# Autodesk Inventor assembly: Swerve-Drivetrain-2
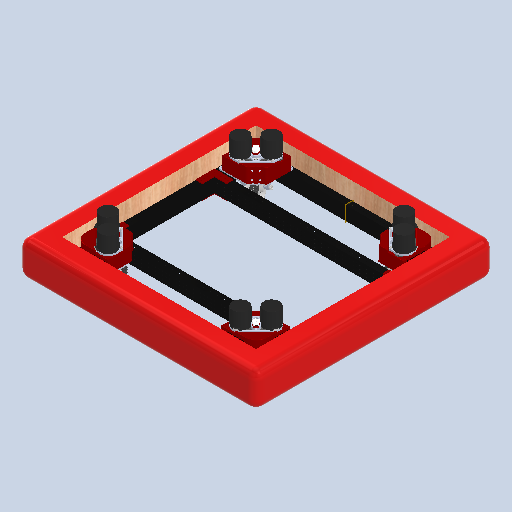
[picture p0: Inventor's stored thumbnail of the model, 512x512]
Saved by Autodesk Inventor 2024 (Build 280153000, 153)
## iProperties
Created: 2024-01-06
Part Number: Swerve-Drivetrain-2
Document SubType Name: Assembly
Designer: rohan
Author: rohan
## Documents named in this file (7)
- C:\Users\5652160\OneDrive - Hillsborough County Public Schools\Robotics\FIRST-Robotics-Competition\Crescendo\Minotaur-Crescendo-Robot\Swerve-Drivetrain.iam
- C:\Users\5652160\OneDrive - Hillsborough County Public Schools\Robotics\FIRST-Robotics-Competition\Crescendo\Minotaur-Crescendo-Robot\Motion\Swerve-Modules\MK3-Swerve-Module-Neos.iam
- C:\Users\5652160\OneDrive - Hillsborough County Public Schools\Robotics\FIRST-Robotics-Competition\Crescendo\Minotaur-Crescendo-Robot\Structure\MAXTube\2024-100-002-Front-Back-Extrusions.ipt
- C:\Users\5652160\OneDrive - Hillsborough County Public Schools\Robotics\FIRST-Robotics-Competition\Crescendo\Minotaur-Crescendo-Robot\Structure\MAXTube\2024-100-001-Left-Right-Extrusions.ipt
- C:\Users\5652160\OneDrive - Hillsborough County Public Schools\Robotics\FIRST-Robotics-Competition\Crescendo\Minotaur-Crescendo-Robot\Structure\MAXTube\2024-100-003-Middle-Extrusions.ipt
- C:\Users\5652160\OneDrive - Hillsborough County Public Schools\Robotics\FIRST-Robotics-Competition\Crescendo\Minotaur-Crescendo-Robot\Structure\Gussets\THRIFYBOT-L-Gusset.ipt
- C:\Users\5652160\OneDrive - Hillsborough County Public Schools\Robotics\FIRST-Robotics-Competition\Crescendo\Minotaur-Crescendo-Robot\Structure\Bumpers.ipt
## Components (23 placed, 6 different names)
1. MK3-Swerve-Module-Neos:1 [sub-assembly] — Mate:75, Mate:80, Mate:81
2. MK3-Swerve-Module-Neos:2 [sub-assembly] — Mate:74, Mate:82, Mate:83
3. MK3-Swerve-Module-Neos:3 [sub-assembly] — Mate:73, Mate:76, Mate:77
4. MK3-Swerve-Module-Neos:4 [sub-assembly] — Mate:72, Mate:78, Mate:79
5. 2024-100-001-Left-Right-Extrusions:1 — Mate:69, Flush:1, Flush:2, Mate:70, Flush:3, Flush:4, Mate:73, Mate:76, Mate:82, Flush:12, Flush:14
6. 2024-100-001-Left-Right-Extrusions:2 — Mate:71, Flush:5, Flush:6, Mate:79, Mate:81, Flush:10, Flush:16, Mate:99
7. 2024-100-002-Front-Back-Extrusions:1 — Mate:70, Flush:3, Flush:4, Mate:72, Mate:77, Mate:78, Mate:84, Mate:85, Mate:88, Mate:89, Flush:13, Flush:15, Flush:30, Mate:96, Flush:32, Mate:97, Flush:33
8. 2024-100-002-Front-Back-Extrusions:2 — Mate:69, Flush:1, Flush:2, Mate:71, Flush:5, Flush:6, Mate:74, Mate:75, Mate:80, Mate:83, Flush:7, Flush:8, Mate:86, Mate:87, Flush:9, Flush:11, Flush:25, Mate:94, Flush:27, Mate:95, Insert:1, Insert:2, Mate:98
9. 2024-100-003-Middle-Extrusions:1 — Mate:85, Flush:7, Flush:26, Flush:29
10. 2024-100-003-Middle-Extrusions:2 — Mate:84, Flush:8, Flush:28, Flush:31
11. THRIFYBOT-L-Gusset:1 — Mate:89, Flush:13, Flush:14
12. THRIFYBOT-L-Gusset:2 — Mate:88, Flush:15, Flush:16
13. THRIFYBOT-L-Gusset:3 — Mate:87, Flush:11, Flush:12
14. THRIFYBOT-L-Gusset:4 — Mate:86, Flush:9, Flush:10
15. THRIFYBOT-L-Gusset:6 — Flush:17, Flush:18, Mate:90, Flush:25, Mate:94, Flush:26, Insert:1
16. THRIFYBOT-L-Gusset:7 — Flush:17, Flush:18, Mate:90
17. THRIFYBOT-L-Gusset:8 — Flush:27, Flush:28, Insert:2
18. THRIFYBOT-L-Gusset:9 — Mate:95
19. THRIFYBOT-L-Gusset:10 — Flush:29, Flush:30
20. THRIFYBOT-L-Gusset:11 — Mate:96
21. THRIFYBOT-L-Gusset:12 — Flush:32, Mate:97
22. THRIFYBOT-L-Gusset:13 — Flush:31
23. Bumpers:1 — Mate:98, Mate:99, Flush:33
## Relationships (66: Flush 33, Mate 31, Insert 2)
- Mate:69: 2024-100-001-Left-Right-Extrusions:1 ↔ 2024-100-002-Front-Back-Extrusions:2
- Flush:1: 2024-100-001-Left-Right-Extrusions:1 ↔ 2024-100-002-Front-Back-Extrusions:2
- Flush:2: 2024-100-001-Left-Right-Extrusions:1 ↔ 2024-100-002-Front-Back-Extrusions:2
- Mate:70: 2024-100-001-Left-Right-Extrusions:1 ↔ 2024-100-002-Front-Back-Extrusions:1
- Flush:3: 2024-100-001-Left-Right-Extrusions:1 ↔ 2024-100-002-Front-Back-Extrusions:1
- Flush:4: 2024-100-001-Left-Right-Extrusions:1 ↔ 2024-100-002-Front-Back-Extrusions:1
- Mate:71: 2024-100-001-Left-Right-Extrusions:2 ↔ 2024-100-002-Front-Back-Extrusions:2
- Flush:5: 2024-100-001-Left-Right-Extrusions:2 ↔ 2024-100-002-Front-Back-Extrusions:2
- Flush:6: 2024-100-001-Left-Right-Extrusions:2 ↔ 2024-100-002-Front-Back-Extrusions:2
- Mate:72: MK3-Swerve-Module-Neos:4 ↔ 2024-100-002-Front-Back-Extrusions:1
- Mate:73: MK3-Swerve-Module-Neos:3 ↔ 2024-100-001-Left-Right-Extrusions:1
- Mate:74: MK3-Swerve-Module-Neos:2 ↔ 2024-100-002-Front-Back-Extrusions:2
- Mate:75: MK3-Swerve-Module-Neos:1 ↔ 2024-100-002-Front-Back-Extrusions:2
- Mate:76: MK3-Swerve-Module-Neos:3 ↔ 2024-100-001-Left-Right-Extrusions:1
- Mate:77: MK3-Swerve-Module-Neos:3 ↔ 2024-100-002-Front-Back-Extrusions:1
- Mate:78: MK3-Swerve-Module-Neos:4 ↔ 2024-100-002-Front-Back-Extrusions:1
- Mate:79: MK3-Swerve-Module-Neos:4 ↔ 2024-100-001-Left-Right-Extrusions:2
- Mate:80: MK3-Swerve-Module-Neos:1 ↔ 2024-100-002-Front-Back-Extrusions:2
- Mate:81: MK3-Swerve-Module-Neos:1 ↔ 2024-100-001-Left-Right-Extrusions:2
- Mate:82: MK3-Swerve-Module-Neos:2 ↔ 2024-100-001-Left-Right-Extrusions:1
- Mate:83: MK3-Swerve-Module-Neos:2 ↔ 2024-100-002-Front-Back-Extrusions:2
- Mate:84: 2024-100-002-Front-Back-Extrusions:1 ↔ 2024-100-003-Middle-Extrusions:2
- Mate:85: 2024-100-002-Front-Back-Extrusions:1 ↔ 2024-100-003-Middle-Extrusions:1
- Flush:7: 2024-100-002-Front-Back-Extrusions:2 ↔ 2024-100-003-Middle-Extrusions:1
- Flush:8: 2024-100-002-Front-Back-Extrusions:2 ↔ 2024-100-003-Middle-Extrusions:2
- Mate:86: 2024-100-002-Front-Back-Extrusions:2 ↔ THRIFYBOT-L-Gusset:4
- Mate:87: 2024-100-002-Front-Back-Extrusions:2 ↔ THRIFYBOT-L-Gusset:3
- Mate:88: 2024-100-002-Front-Back-Extrusions:1 ↔ THRIFYBOT-L-Gusset:2
- Mate:89: 2024-100-002-Front-Back-Extrusions:1 ↔ THRIFYBOT-L-Gusset:1
- Flush:9: 2024-100-002-Front-Back-Extrusions:2 ↔ THRIFYBOT-L-Gusset:4
- Flush:10: 2024-100-001-Left-Right-Extrusions:2 ↔ THRIFYBOT-L-Gusset:4
- Flush:11: 2024-100-002-Front-Back-Extrusions:2 ↔ THRIFYBOT-L-Gusset:3
- Flush:12: 2024-100-001-Left-Right-Extrusions:1 ↔ THRIFYBOT-L-Gusset:3
- Flush:13: 2024-100-002-Front-Back-Extrusions:1 ↔ THRIFYBOT-L-Gusset:1
- Flush:14: 2024-100-001-Left-Right-Extrusions:1 ↔ THRIFYBOT-L-Gusset:1
- Flush:15: 2024-100-002-Front-Back-Extrusions:1 ↔ THRIFYBOT-L-Gusset:2
- Flush:16: 2024-100-001-Left-Right-Extrusions:2 ↔ THRIFYBOT-L-Gusset:2
- Flush:17: THRIFYBOT-L-Gusset:6 ↔ THRIFYBOT-L-Gusset:7
- Flush:18: THRIFYBOT-L-Gusset:6 ↔ THRIFYBOT-L-Gusset:7
- Mate:90 (50.8 mm): THRIFYBOT-L-Gusset:6 ↔ THRIFYBOT-L-Gusset:7
- [Flush]: THRIFYBOT-L-Gusset:8 ↔ THRIFYBOT-L-Gusset:9
- [Flush]: THRIFYBOT-L-Gusset:8 ↔ THRIFYBOT-L-Gusset:9
- [Mate] (50.8 mm): THRIFYBOT-L-Gusset:8 ↔ THRIFYBOT-L-Gusset:9
- [Flush]: THRIFYBOT-L-Gusset:10 ↔ THRIFYBOT-L-Gusset:11
- [Flush]: THRIFYBOT-L-Gusset:10 ↔ THRIFYBOT-L-Gusset:11
- [Mate] (50.8 mm): THRIFYBOT-L-Gusset:10 ↔ THRIFYBOT-L-Gusset:11
- [Flush]: THRIFYBOT-L-Gusset:12 ↔ THRIFYBOT-L-Gusset:13
- [Flush]: THRIFYBOT-L-Gusset:12 ↔ THRIFYBOT-L-Gusset:13
- [Mate] (50.8 mm): THRIFYBOT-L-Gusset:12 ↔ THRIFYBOT-L-Gusset:13
- Flush:25: 2024-100-002-Front-Back-Extrusions:2 ↔ THRIFYBOT-L-Gusset:6
- Mate:94: 2024-100-002-Front-Back-Extrusions:2 ↔ THRIFYBOT-L-Gusset:6
- Flush:26: 2024-100-003-Middle-Extrusions:1 ↔ THRIFYBOT-L-Gusset:6
- Flush:27: 2024-100-002-Front-Back-Extrusions:2 ↔ THRIFYBOT-L-Gusset:8
- Mate:95: 2024-100-002-Front-Back-Extrusions:2 ↔ THRIFYBOT-L-Gusset:9
- Flush:28: 2024-100-003-Middle-Extrusions:2 ↔ THRIFYBOT-L-Gusset:8
- Flush:29: 2024-100-003-Middle-Extrusions:1 ↔ THRIFYBOT-L-Gusset:10
- Flush:30: 2024-100-002-Front-Back-Extrusions:1 ↔ THRIFYBOT-L-Gusset:10
- Mate:96: 2024-100-002-Front-Back-Extrusions:1 ↔ THRIFYBOT-L-Gusset:11
- Flush:31: 2024-100-003-Middle-Extrusions:2 ↔ THRIFYBOT-L-Gusset:13
- Flush:32: 2024-100-002-Front-Back-Extrusions:1 ↔ THRIFYBOT-L-Gusset:12
- Mate:97: 2024-100-002-Front-Back-Extrusions:1 ↔ THRIFYBOT-L-Gusset:12
- Insert:1: 2024-100-002-Front-Back-Extrusions:2 ↔ THRIFYBOT-L-Gusset:6
- Insert:2: 2024-100-002-Front-Back-Extrusions:2 ↔ THRIFYBOT-L-Gusset:8
- Mate:98: 2024-100-002-Front-Back-Extrusions:2 ↔ Bumpers:1
- Mate:99: 2024-100-001-Left-Right-Extrusions:2 ↔ Bumpers:1
- Flush:33 (63.5 mm): 2024-100-002-Front-Back-Extrusions:1 ↔ Bumpers:1
## Named parameters: d247_d244 = 0 mm, d248_d245 = 0 mm, d249_d246 = 50.8 mm, d250_d244 = 0 mm, d251_d245 = 0 mm, d252_d246 = 50.8 mm, d253_d244 = 0 mm, d254_d245 = 0 mm, d255_d246 = 50.8 mm
